# Autodesk Inventor assembly: Beamerscope_r4
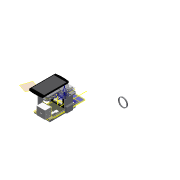
[picture p0: Inventor's stored thumbnail of the model, 180x180]
Saved by Autodesk Inventor 2016 (Build 200138000, 138)
## iProperties
Created: 2017-01-03
Part Number: Beamerscope_r4
Material: Generisch
Document SubType Name: Assembly
Designer: diederichbenedict
Author: diederichbenedict
## Documents named in this file (19)
- C:\Users\diederichbenedict\Documents\Inventor\Beamerscope_r4\Beamerscope_r4.iam
- C:\Users\diederichbenedict\Documents\Inventor\Beamerscope_r4\05_Case_Bottom.ipt
- C:\Users\diederichbenedict\Documents\Inventor\Beamerscope_r4\06_Case_Upper.ipt
- C:\Users\diederichbenedict\Documents\Inventor\Beamerscope_r4\27_Focus_Knob.ipt
- C:\Users\diederichbenedict\Documents\Inventor\Beamerscope_r4\28_Z_Stage.ipt
- C:\Users\diederichbenedict\Documents\Inventor\Beamerscope_r4\00_Stange.ipt
- C:\Users\diederichbenedict\Documents\Inventor\Beamerscope_r4\DIN EN ISO 4036 - M6.ipt
- C:\Users\diederichbenedict\Documents\Inventor\Beamerscope_r4\DIN 6912 - M6 x 20.ipt
- C:\Users\diederichbenedict\Documents\Inventor\Beamerscope_r4\LED.iam
- C:\Users\diederichbenedict\Documents\Inventor\Beamerscope_r4\Lensholder_Assembly.iam
- C:\Users\diederichbenedict\Documents\Inventor\Beamerscope_r4\Mutter.ipt
- C:\Users\diederichbenedict\Documents\Inventor\Beamerscope_r4\Nexus 5.ipt
- C:\Users\diederichbenedict\Documents\Inventor\Beamerscope_r4\Projector_PCB.iam
- C:\Users\diederichbenedict\Documents\Inventor\Beamerscope_r4\RJMP_01_08_2.ipt
- C:\Users\diederichbenedict\Documents\Inventor\Beamerscope_r4\26_Lensholder_Aspheric_right.ipt
- C:\Users\diederichbenedict\Documents\Inventor\Beamerscope_r4\27_Nut.ipt
- C:\Users\diederichbenedict\Documents\Inventor\Beamerscope_r4\ACL3026U-Step.ipt
- C:\Users\diederichbenedict\Documents\Inventor\Beamerscope_r4\11_Objektträger.ipt
- C:\Users\diederichbenedict\Documents\Inventor\Beamerscope_r4\11_Smartphone_Platform.ipt
## Components (20 placed, 18 different names)
1. 05_Case_Bottom:1 — Passend:1, Einfügen:1, Einfügen:2, Einfügen:3, Einfügen:4, Passend:3, Passend:4, Fluchtend:1
2. 06_Case_Upper:1 — Einfügen:3, Einfügen:4, Einfügen:5, Einfügen:6, Einfügen:7, Einfügen:8, Einfügen:10, Einfügen:11, Einfügen:13, Fluchtend:2, Fluchtend:3
3. 27_Focus_Knob:1 — Einfügen:8, Winkel:1
4. 28_Z_Stage:1 — Einfügen:12, Passend:2, Passend:5, Winkel:2
5. 00_Stange:1 — Einfügen:5
6. DIN EN ISO 4036 M6:1 — Einfügen:9, Winkel:1
7. DIN 6912 M6 x 20:1 — Einfügen:7, Einfügen:9
8. LED:1 [sub-assembly] — Passend:3, Passend:4, Fluchtend:1
9. Lensholder_Assembly:1 [sub-assembly]
10. Mutter:1
11. Nexus 5:1 — Einfügen:16, Winkel:2
12. Projector_PCB:1 [sub-assembly] — Einfügen:1, Einfügen:2
13. RJMP_01_08_2:1 — Einfügen:10
14. 26_Lensholder_Aspheric_right:1 — Einfügen:14, Einfügen:15, Einfügen:16
15. 27_Nut:1 — Einfügen:13, Einfügen:14
16. ACL3026U-Step:1 — Einfügen:15
17. 11_Objektträger:1 — Passend:5
18. 00_Stange:2 — Einfügen:6, Passend:2
19. RJMP_01_08_2:2 — Einfügen:11, Einfügen:12
20. 11_Smartphone_Platform:1 — Fluchtend:2, Fluchtend:3
## Relationships (26: Insert 16, Mate 5, Flush 3, Angle 2)
- Passend:1 [Mate]: 05_Case_Bottom:1
- Einfügen:1 [Insert]: 05_Case_Bottom:1 ↔ Projector_PCB:1
- Einfügen:2 [Insert]: 05_Case_Bottom:1 ↔ Projector_PCB:1
- Einfügen:3 [Insert]: 05_Case_Bottom:1 ↔ 06_Case_Upper:1
- Einfügen:4 [Insert]: 05_Case_Bottom:1 ↔ 06_Case_Upper:1
- Einfügen:5 [Insert]: 06_Case_Upper:1 ↔ 00_Stange:1
- Einfügen:6 [Insert]: 06_Case_Upper:1 ↔ 00_Stange:2
- Einfügen:7 [Insert]: 06_Case_Upper:1 ↔ DIN 6912 M6 x 20:1
- Einfügen:8 [Insert] (-4 mm): 06_Case_Upper:1 ↔ 27_Focus_Knob:1
- Einfügen:9 [Insert] (-12 mm): DIN EN ISO 4036 M6:1 ↔ DIN 6912 M6 x 20:1
- Winkel:1 [Angle] (0 deg): 27_Focus_Knob:1 ↔ DIN EN ISO 4036 M6:1
- Einfügen:10 [Insert] (2 mm): 06_Case_Upper:1 ↔ RJMP_01_08_2:1
- Einfügen:11 [Insert] (2 mm): 06_Case_Upper:1 ↔ RJMP_01_08_2:2
- Einfügen:12 [Insert] (-2 mm): 28_Z_Stage:1 ↔ RJMP_01_08_2:2
- Passend:2 [Mate]: 28_Z_Stage:1 ↔ 00_Stange:2
- Passend:3 [Mate]: 05_Case_Bottom:1 ↔ LED:1
- Passend:4 [Mate]: 05_Case_Bottom:1 ↔ LED:1
- Fluchtend:1 [Flush]: 05_Case_Bottom:1 ↔ LED:1
- Einfügen:13 [Insert]: 06_Case_Upper:1 ↔ 27_Nut:1
- Einfügen:14 [Insert] (-15 mm): 26_Lensholder_Aspheric_right:1 ↔ 27_Nut:1
- Einfügen:15 [Insert] (-2 mm): 26_Lensholder_Aspheric_right:1 ↔ ACL3026U-Step:1
- Passend:5 [Mate]: 28_Z_Stage:1 ↔ 11_Objektträger:1
- Einfügen:16 [Insert] (10 mm): Nexus 5:1 ↔ 26_Lensholder_Aspheric_right:1
- Winkel:2 [Angle] (180 deg): 28_Z_Stage:1 ↔ Nexus 5:1
- Fluchtend:2 [Flush]: 06_Case_Upper:1 ↔ 11_Smartphone_Platform:1
- Fluchtend:3 [Flush]: 06_Case_Upper:1 ↔ 11_Smartphone_Platform:1
